# Autodesk Inventor assembly: 4in Performance Hex Bore nitrile 2012 Redesign
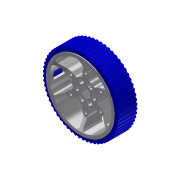
[picture p0: Inventor's stored thumbnail of the model, 180x180]
Saved by Autodesk Inventor 2013 (Build 170138000, 138)
## iProperties
Created: 2013-12-17
Part Number: 4in Performance Hex Bore nitrile 2012 Redesign
Document SubType Name: Assembly
Designer: Nemo
Author: Nemo
## Documents named in this file (3)
- H:\Nemo\Documents\Robotics\COTS Parts\Wheels\AndyMark Performance Wheels\4in Performance Hex Bore nitrile 2012 Redesign.iam
- H:\Nemo\Documents\Robotics\COTS Parts\Wheels\AndyMark Performance Wheels\Components\4in Performance Hex 2012 Redesign.ipt
- H:\Nemo\Documents\Robotics\COTS Parts\Wheels\Tread\Nitrile Tread.ipt
## Components (2 placed, 2 different names)
1. 4in Performance Hex 2012 Redesign:1 — Mate:1, Mate:2
2. Nitrile Tread:1 — Mate:1, Mate:2
## Relationships (2: Mate 2)
- Mate:1: 4in Performance Hex 2012 Redesign:1 ↔ Nitrile Tread:1
- Mate:2: 4in Performance Hex 2012 Redesign:1 ↔ Nitrile Tread:1
